# Autodesk Inventor assembly: dIII
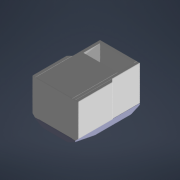
[picture p0: Inventor's stored thumbnail of the model, 180x180]
Saved by Autodesk Inventor 2022 (Build 260153000, 153)
## iProperties
Created: 2022-03-30
Part Number: dIII
Document SubType Name: Assembly
Designer: Kalugin_a
Author: Kalugin_a
## Documents named in this file (10)
- D:\GitHUB\MELAS\Workspace\DIII\dIII.iam
- D:\GitHUB\MELAS\Workspace\DIII\Front.ipt
- D:\GitHUB\MELAS\Workspace\DIII\side_A.ipt
- D:\GitHUB\MELAS\Workspace\DIII\side_A1.ipt
- D:\GitHUB\MELAS\Workspace\DIII\self.ipt
- D:\GitHUB\MELAS\Workspace\DIII\Top-Bott.ipt
- D:\GitHUB\MELAS\Workspace\DIII\double_side_A.ipt
- D:\GitHUB\MELAS\Workspace\DIII\double_side_A1.ipt
- D:\GitHUB\MELAS\Workspace\DIII\back.ipt
- D:\GitHUB\MELAS\Workspace\DIII\midwall.ipt
## Components (10 placed, 9 different names)
1. Front:1 — Жесткий:1, Жесткий:2, Совмещение:3, Совмещение:5
2. side_A:1 — Жесткий:2, Совмещение:1, Совмещение:2, Совмещение:4, Совмещение:8, Совмещение:9
3. side_A1:1 — Жесткий:1, Совмещение:6, Совмещение:7, Совмещение:11
4. self:1 — Совмещение:1, Совмещение:12, Совмещение:14
5. Top-Bott:1 — Совмещение:2, Совмещение:3
6. Top-Bott:2 — Совмещение:4, Совмещение:5, Совмещение:10
7. double_side_A:1 — Совмещение:6, Совмещение:7
8. double_side_A1:1 — Совмещение:8, Совмещение:9
9. back:1 — Совмещение:10, Совмещение:11, Совмещение:12
10. midwall:1 — Совмещение:14
## Relationships (15: Mate 13, WeldJoint 2)
- Жесткий:1 [WeldJoint]: Front:1 ↔ side_A1:1
- Жесткий:2 [WeldJoint]: Front:1 ↔ side_A:1
- Совмещение:1 [Mate]: side_A:1 ↔ self:1
- Совмещение:2 [Mate]: side_A:1 ↔ Top-Bott:1
- Совмещение:3 [Mate]: Front:1 ↔ Top-Bott:1
- Совмещение:4 [Mate]: side_A:1 ↔ Top-Bott:2
- Совмещение:5 [Mate]: Front:1 ↔ Top-Bott:2
- Совмещение:6 [Mate]: side_A1:1 ↔ double_side_A:1
- Совмещение:7 [Mate]: side_A1:1 ↔ double_side_A:1
- Совмещение:8 [Mate]: side_A:1 ↔ double_side_A1:1
- Совмещение:9 [Mate]: side_A:1 ↔ double_side_A1:1
- Совмещение:10 [Mate]: Top-Bott:2 ↔ back:1
- Совмещение:11 [Mate]: side_A1:1 ↔ back:1
- Совмещение:12 [Mate]: self:1 ↔ back:1
- Совмещение:14 [Mate]: self:1 ↔ midwall:1
